# Autodesk Inventor assembly: 20-004
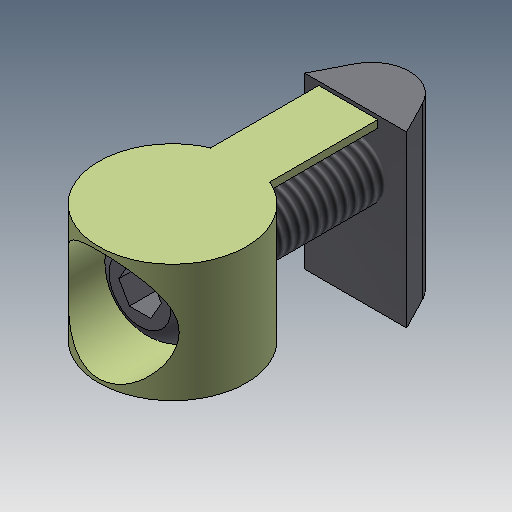
[picture p0: Inventor's stored thumbnail of the model, 512x512]
Saved by Autodesk Inventor 2018.3 (Build 223284000, 284)
## iProperties
Created: 2004-10-14
Part Number: 20-004
Document SubType Name: Assembly
Designer: Autodesk, Inc.
Manufacturer: Standard
Standards Organization: Custom
Description: UNIVERSAL FASTENER SET, 40 SERIES
Catalog Web Link: http://www.parker.com/ead/cm1.asp?cmid=809
Vendor: PARKER IPS
Mass: 43.7862 g
Surface Area: 46.6491 cm^2
Volume: 6.24795 cm^3
Density: 7.00809 g/cm^3
CAGE: 1LJX3
Dept. ID: Product Design
Description #2: ---
Finish #1: ---
Finish #2: ---
Material ID: ---
Project Number: ---
Author: Autodesk, Inc.
## Documents named in this file (7)
- C:\AVAInvAPI\Workspace\Test Station\Components\20-004.iam
- C:\AVAInvAPI\Workspace\Test Station\Components\20-004Z1.ipt
- C:\AVAInvAPI\Workspace\Test Station\Components\24-130-8.ipt
- C:\AVAInvAPI\Workspace\Test Station\Components\20-058.ipt
- C:\workfolder\Extra Samples\Models\Test Station\Library\Parker - IPS\Fastners\2X-YYY Universal Fastner.ipt
- C:\workfolder\Extra Samples\Models\Test Station\Library\Parker - IPS\Fastners\2X-YYY-ZZ IPS Screws.ipt
- C:\workfolder\Extra Samples\Models\Test Station\Library\Parker - IPS\Fastners\20-XXX TSlot Nuts.ipt
## Components (3 placed, 3 different names)
1. 20-004Z1:1 — Mate:1, Mate:2, Mate:4, Angle:1
2. 24-130-8:1 — Mate:1, Mate:2, Mate:3
3. 20-058:1 — Mate:3, Mate:4, Angle:1
## Relationships (5: Mate 4, Angle 1)
- Mate:1: 20-004Z1:1 ↔ 24-130-8:1
- Mate:2: 20-004Z1:1 ↔ 24-130-8:1
- Mate:3: 24-130-8:1 ↔ 20-058:1
- Mate:4 (1 mm): 20-004Z1:1 ↔ 20-058:1
- Angle:1 (0 deg): 20-004Z1:1 ↔ 20-058:1
